# Autodesk Inventor assembly: rocker_bogie_right
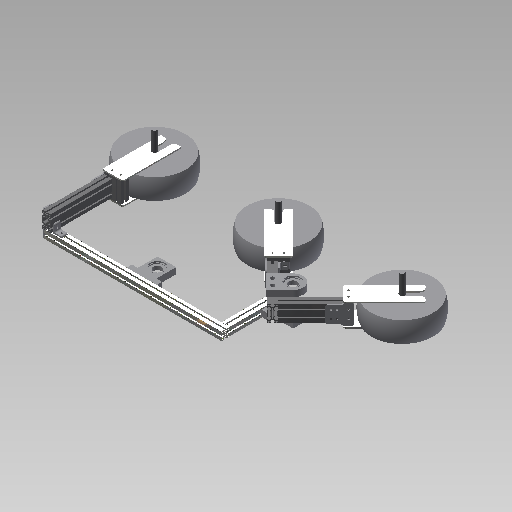
[picture p0: Inventor's stored thumbnail of the model, 512x512]
Saved by Autodesk Inventor 2021.2 (Build 252289000, 289)
## iProperties
Created: 2021-05-27
Part Number: rocker_bogie_right
Document SubType Name: Assembly
Designer: gisen
Author: gisen
## Documents named in this file (8)
- C:\Users\gisen\workspace\beetle_inventor_model\suspension\rocker_bogie_right.iam
- C:\Users\gisen\workspace\beetle_inventor_model\suspension\rocker_right.iam
- C:\Users\gisen\workspace\beetle_inventor_model\suspension\bogie_right.iam
- C:\Users\gisen\workspace\beetle_inventor_model\suspension\AFS-2020-4-150_right.ipt
- C:\Users\gisen\workspace\beetle_inventor_model\suspension\BSHKSA6904ZZ-40\BSHKSA6904ZZ-40_right.iam
- C:\Users\gisen\workspace\beetle_inventor_model\suspension\AFS-2020-4-430_right.ipt
- C:\Users\gisen\workspace\beetle_inventor_model\suspension\M4L_right.ipt
- C:\Users\gisen\workspace\beetle_inventor_model\suspension\rocker_bogie_mount_right.ipt
## Components (9 placed, 4 different names)
1. rocker_right:1 [sub-assembly] — 角度:1, フラッシュ:2, メイト:1, メイト:3, フラッシュ:1, メイト:13, メイト:11, メイト:14, メイト:18, 対称度:1
2. bogie_right:1 [sub-assembly] — フラッシュ:3, メイト:4, メイト:3, フラッシュ:1, メイト:9, メイト:6
3. Part1:1 — 角度:2, メイト:9, フラッシュ:9, メイト:7, メイト:5, メイト:10, フラッシュ:5, フラッシュ:4
4. BSHKSA6904ZZ-40_right:1 [sub-assembly] — フラッシュ:9, メイト:7, メイト:6, メイト:5
5. Part1:2 — メイト:10, フラッシュ:5, フラッシュ:4, メイト:12, フラッシュ:10, メイト:15, メイト:17, メイト:16, メイト:21, メイト:20, メイト:19, 対称度:1
6. Part1:3 — メイト:13, メイト:12, メイト:11
7. Part1:4 — フラッシュ:10, メイト:15, メイト:14
8. Part1:5 — メイト:18, メイト:17, メイト:16
9. BSHKSA6904ZZ-40_right:2 [sub-assembly] — メイト:21, メイト:20, メイト:19, メイト:22
## Relationships (30: Mate 20, Flush 7, Angle 2, Symmetry 1)
- 角度:1 [Angle] (180 deg): rocker_right:1
- フラッシュ:2 [Flush]: rocker_right:1
- メイト:1 [Mate]: rocker_right:1
- フラッシュ:3 [Flush]: bogie_right:1
- メイト:4 [Mate]: bogie_right:1
- メイト:3 [Mate] (300 mm): rocker_right:1 ↔ bogie_right:1
- フラッシュ:1 [Flush]: rocker_right:1 ↔ bogie_right:1
- 角度:2 [Angle] (180 deg): Part1:1
- メイト:9 [Mate] (3 mm): bogie_right:1 ↔ Part1:1
- フラッシュ:9 [Flush]: Part1:1 ↔ BSHKSA6904ZZ-40_right:1
- メイト:7 [Mate] (-10 mm): Part1:1 ↔ BSHKSA6904ZZ-40_right:1
- メイト:6 [Mate]: bogie_right:1 ↔ BSHKSA6904ZZ-40_right:1
- メイト:5 [Mate]: Part1:1 ↔ BSHKSA6904ZZ-40_right:1
- メイト:10 [Mate]: Part1:1 ↔ Part1:2
- フラッシュ:5 [Flush]: Part1:1 ↔ Part1:2
- フラッシュ:4 [Flush]: Part1:1 ↔ Part1:2
- メイト:13 [Mate] (-10 mm): rocker_right:1 ↔ Part1:3
- メイト:12 [Mate]: Part1:2 ↔ Part1:3
- メイト:11 [Mate]: rocker_right:1 ↔ Part1:3
- フラッシュ:10 [Flush]: Part1:2 ↔ Part1:4
- メイト:15 [Mate]: Part1:2 ↔ Part1:4
- メイト:14 [Mate]: rocker_right:1 ↔ Part1:4
- メイト:18 [Mate]: rocker_right:1 ↔ Part1:5
- メイト:17 [Mate] (-10 mm): Part1:2 ↔ Part1:5
- メイト:16 [Mate]: Part1:2 ↔ Part1:5
- メイト:21 [Mate] (-10 mm): Part1:2 ↔ BSHKSA6904ZZ-40_right:2
- メイト:20 [Mate] (-10 mm): Part1:2 ↔ BSHKSA6904ZZ-40_right:2
- メイト:19 [Mate]: Part1:2 ↔ BSHKSA6904ZZ-40_right:2
- メイト:22 [Mate]: BSHKSA6904ZZ-40_right:2
- 対称度:1 [Symmetry]: rocker_right:1 ↔ Part1:2
